# Autodesk Inventor assembly: Assembly Version 2.1
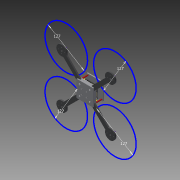
[picture p0: Inventor's stored thumbnail of the model, 180x180]
Saved by Autodesk Inventor 2015 (Build 190159000, 159)
## iProperties
Created: 2017-02-15
Part Number: Assembly Version 2.1
Document SubType Name: Assembly
Designer: Hampus
Author: Hampus
## Documents named in this file (11)
- C:\Users\Hampus.Hampus-Dator\Desktop\Gymnasiearbete\Version 2.0\Assembly Version 2.1.iam
- C:\Users\Hampus.Hampus-Dator\Desktop\Gymnasiearbete\Version 2.0\Bot 2.1.ipt
- C:\Users\Hampus.Hampus-Dator\Desktop\Gymnasiearbete\Version 2.0\Arm2.ipt
- C:\Users\Hampus.Hampus-Dator\Desktop\Gymnasiearbete\Version 2.0\Naze32 Acro.ipt
- C:\Users\Hampus.Hampus-Dator\Desktop\Gymnasiearbete\Version 2.0\PDB 2.1.ipt
- C:\Users\Hampus.Hampus-Dator\Desktop\Gymnasiearbete\Version 2.0\Standoff.ipt
- C:\Users\Hampus.Hampus-Dator\Desktop\Gymnasiearbete\Version 2.0\Alu M3x20.ipt
- C:\Users\Hampus.Hampus-Dator\Desktop\Gymnasiearbete\Version 2.0\M3x13.ipt
- C:\Users\Hampus.Hampus-Dator\Desktop\Gymnasiearbete\Version 2.0\Topp 2.1.ipt
- C:\Users\Hampus.Hampus-Dator\Desktop\Gymnasiearbete\Version 2.0\Batt_Plate_FPV.ipt
- C:\Users\Hampus.Hampus-Dator\Desktop\Gymnasiearbete\Version 2.0\M3x7.ipt
## Components (37 placed, 10 different names)
1. Bot 2.1:1 — Insert:1, Rigid:1, Rigid:2, Rigid:3, Insert:7, Insert:8, Insert:9, Insert:10
2. Arm2:1 — Insert:1
3. Arm2:2 — Rigid:1, Insert:2
4. Arm2:3 — Rigid:3
5. Arm2:4 — Rigid:2
6. Naze32 Acro:1 — Insert:24
7. Standoff:1 — Insert:23, Insert:24
8. Standoff:2 — Insert:17
9. Standoff:3 — Insert:22
10. Standoff:4 — Insert:18
11. Standoff:5 — Insert:21
12. Standoff:6 — Insert:20
13. Standoff:7 — Insert:16
14. Standoff:8 — Insert:15, Insert:19
15. Alu M3x20:1 — Insert:25
16. Alu M3x20:2 — Insert:26
17. Alu M3x20:3 — Insert:28, Insert:29
18. Alu M3x20:4 — Insert:27
19. M3x13:1 — Insert:14
20. M3x13:2 — Insert:12
21. M3x13:3 — Insert:13
22. M3x13:4 — Insert:11
23. M3x13:5 — Insert:10
24. M3x13:6 — Insert:9
25. M3x13:7 — Insert:8
26. M3x13:8 — Insert:7
27. M3x13:9 — Insert:4
28. M3x13:10 — Insert:5
29. M3x13:11 — Insert:6
30. M3x13:12 — Insert:3
31. Topp 2.1:1 — Insert:2, Insert:3, Insert:4, Insert:5, Insert:6, Insert:11, Insert:12, Insert:13, Insert:14, Insert:15, Insert:16, Insert:17, Insert:18, Insert:25, Insert:26, Insert:27, Insert:28
32. PDB 2.1:1 — Insert:19, Insert:20, Insert:21, Insert:22, Insert:23
33. Batt_Plate_FPV:1 — Insert:29, Insert:30, Insert:31, Insert:32, Insert:33
34. M3x7:1 — Insert:33
35. M3x7:2 — Insert:31
36. M3x7:3 — Insert:30
37. M3x7:4 — Insert:32
## Relationships (36: Insert 33, WeldJoint 3)
- Insert:1: Bot 2.1:1 ↔ Arm2:1
- Rigid:1 [WeldJoint]: Bot 2.1:1 ↔ Arm2:2
- Rigid:2 [WeldJoint]: Bot 2.1:1 ↔ Arm2:4
- Rigid:3 [WeldJoint]: Bot 2.1:1 ↔ Arm2:3
- Insert:2: Arm2:2 ↔ Topp 2.1:1
- Insert:3: M3x13:12 ↔ Topp 2.1:1
- Insert:4: M3x13:9 ↔ Topp 2.1:1
- Insert:5: M3x13:10 ↔ Topp 2.1:1
- Insert:6: M3x13:11 ↔ Topp 2.1:1
- Insert:7: Bot 2.1:1 ↔ M3x13:8
- Insert:8: Bot 2.1:1 ↔ M3x13:7
- Insert:9: Bot 2.1:1 ↔ M3x13:6
- Insert:10: Bot 2.1:1 ↔ M3x13:5
- Insert:11: M3x13:4 ↔ Topp 2.1:1
- Insert:12: M3x13:2 ↔ Topp 2.1:1
- Insert:13: M3x13:3 ↔ Topp 2.1:1
- Insert:14: M3x13:1 ↔ Topp 2.1:1
- Insert:15: Standoff:8 ↔ Topp 2.1:1
- Insert:16: Standoff:7 ↔ Topp 2.1:1
- Insert:17: Standoff:2 ↔ Topp 2.1:1
- Insert:18: Standoff:4 ↔ Topp 2.1:1
- Insert:19: Standoff:8 ↔ PDB 2.1:1
- Insert:20: Standoff:6 ↔ PDB 2.1:1
- Insert:21: Standoff:5 ↔ PDB 2.1:1
- Insert:22: Standoff:3 ↔ PDB 2.1:1
- Insert:23: Standoff:1 ↔ PDB 2.1:1
- Insert:24: Naze32 Acro:1 ↔ Standoff:1
- Insert:25: Alu M3x20:1 ↔ Topp 2.1:1
- Insert:26: Alu M3x20:2 ↔ Topp 2.1:1
- Insert:27: Alu M3x20:4 ↔ Topp 2.1:1
- Insert:28: Alu M3x20:3 ↔ Topp 2.1:1
- Insert:29: Alu M3x20:3 ↔ Batt_Plate_FPV:1
- Insert:30: Batt_Plate_FPV:1 ↔ M3x7:3
- Insert:31: Batt_Plate_FPV:1 ↔ M3x7:2
- Insert:32: Batt_Plate_FPV:1 ↔ M3x7:4
- Insert:33: Batt_Plate_FPV:1 ↔ M3x7:1
